# Autodesk Inventor assembly: ASY MSC 400 Accsess hatch
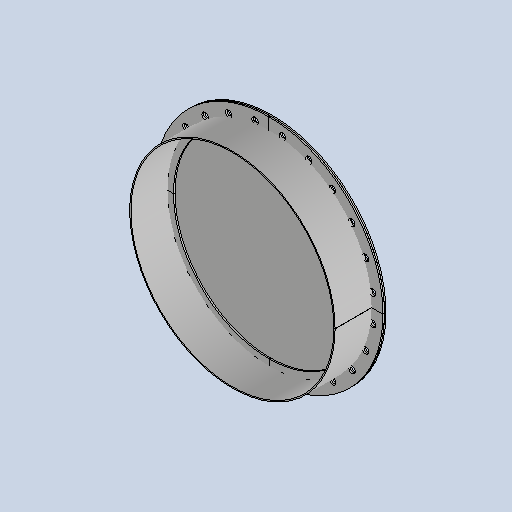
[picture p0: Inventor's stored thumbnail of the model, 512x512]
Saved by Autodesk Inventor 2025 (Build 290162010, 162A)
## iProperties
Created: 2024-09-04
Part Number: ASY MSC 400 Accsess hatch
Document SubType Name: Assembly
Designer: admin
Stock Number: ASY МОО 400 люк доступа
Author: admin
## Documents named in this file (6)
- C:\Users\pokla\Documents\Inventor\Manturovo2\ASY MSC 400 Accsess hatch.iam
- C:\Users\pokla\Documents\Inventor\Manturovo2\MSC 402 ring.ipt
- C:\Users\pokla\Documents\Inventor\Manturovo2\MSC 403 flange 500.ipt
- C:\Users\pokla\Documents\Inventor\Manturovo2\MSC 404 flange cover 500.ipt
- C:\Users\pokla\Documents\Inventor\Manturovo2\MSC 405 flange cover ring 500.ipt
- C:\Users\pokla\Documents\Inventor\Manturovo2\MSC 406 flange cover plate 500.ipt
## Components (19 placed, 5 different names)
1. MSC 402 ring.ipt:1
2. MSC 403 flange 500.ipt:1
3. MSC 403 flange 500.ipt:2
4. MSC 403 flange 500.ipt:3
5. MSC 403 flange 500.ipt:4
6. MSC 404 flange cover 500.ipt:1
7. MSC 405 flange cover ring 500.ipt:1
8. MSC 406 flange cover plate 500.ipt:1
9. MSC 406 flange cover plate 500.ipt:2
10. MSC 406 flange cover plate 500.ipt:3
11. MSC 406 flange cover plate 500.ipt:4
12. MSC 406 flange cover plate 500.ipt:5
13. MSC 406 flange cover plate 500.ipt:6
14. MSC 406 flange cover plate 500.ipt:7
15. MSC 406 flange cover plate 500.ipt:8
16. MSC 406 flange cover plate 500.ipt:9
17. MSC 406 flange cover plate 500.ipt:10
18. MSC 406 flange cover plate 500.ipt:11
19. MSC 406 flange cover plate 500.ipt:12
## Component patterns: (12 elements, first: MSC 406 flange cover plate 500.ipt:1)
## Relationships (10: WeldJoint 5, Mate 3, RevoluteJoint 1, Tangent 1)
- [WeldJoint]: MSC 403 flange 500.ipt:1 ↔ MSC 403 flange 500.ipt:2
- [WeldJoint]: MSC 403 flange 500.ipt:2 ↔ MSC 403 flange 500.ipt:3
- [WeldJoint]: MSC 403 flange 500.ipt:3 ↔ MSC 403 flange 500.ipt:4
- [RevoluteJoint]: MSC 403 flange 500.ipt:4 ↔ MSC 404 flange cover 500.ipt:1
- [Mate]: MSC 403 flange 500.ipt:3 ↔ MSC 404 flange cover 500.ipt:1
- [WeldJoint]: MSC 404 flange cover 500.ipt:1 ↔ MSC 405 flange cover ring 500.ipt:1
- [Mate]: MSC 404 flange cover 500.ipt:1 ↔ MSC 406 flange cover plate 500.ipt:1
- [Mate]: MSC 405 flange cover ring 500.ipt:1 ↔ MSC 406 flange cover plate 500.ipt:1
- [Tangent]: MSC 405 flange cover ring 500.ipt:1 ↔ MSC 406 flange cover plate 500.ipt:1
- [WeldJoint]: MSC 402 ring.ipt:1 ↔ MSC 403 flange 500.ipt:2
